# Autodesk Inventor assembly: welding-desk
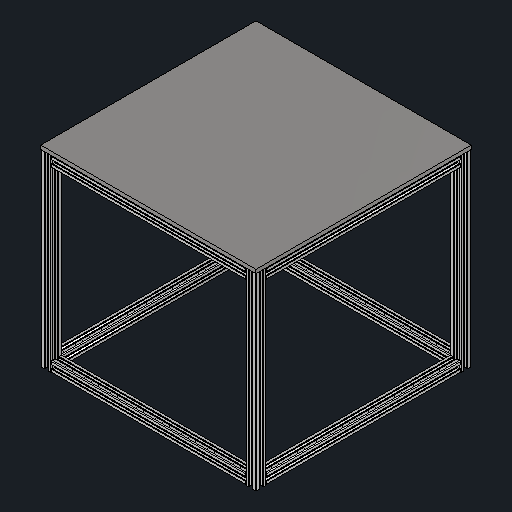
[picture p0: Inventor's stored thumbnail of the model, 512x512]
Saved by Autodesk Inventor 2026 (Build 300175050, 175E)
## iProperties
Created: 2026-01-15
Part Number: welding-desk
Document SubType Name: Assembly
Designer: queezz
Author: queezz
## Documents named in this file (5)
- C:\Users\queezz\Dropbox\Drawings\PIHTI\Desks\welding-desk.iam
- C:\Users\queezz\Dropbox\Drawings\PIHTI\Desks\welding-desk-top.ipt
- C:\Users\queezz\Dropbox\Drawings\PIHTI\ContentCenter\Aluminium-profiles\Al-profile-20x20.ipt
- C:\Users\queezz\Dropbox\Drawings\PIHTI\ContentCenter\Aluminium-profiles\Al-profile-20x20\Al-profile-20x20-360.ipt
- C:\Users\queezz\Dropbox\Drawings\PIHTI\ContentCenter\Aluminium-profiles\Al-profile-20x20\Al-profile-20x20-350.ipt
## Components (13 placed, 3 different names)
1. welding-desk-top:1 — Mate:1, Mate:2, Mate:3, Mate:4, Flush:1, Flush:2, Flush:3, Flush:4, Flush:5, Flush:6, Flush:7, Flush:8
2. Al-profile-20x20-360:1 — Mate:6, Flush:9, Flush:14, Flush:15, Flush:16
3. Al-profile-20x20-360:2 — Mate:8, Flush:11, Flush:13, Flush:14
4. Al-profile-20x20-360:3 — Mate:7, Flush:12, Flush:13
5. Al-profile-20x20-360:4 — Mate:5, Flush:10, Flush:15
6. Al-profile-20x20-360:5 — Mate:10, Flush:22, Flush:23
7. Al-profile-20x20-360:6 — Mate:12, Flush:17, Flush:20
8. Al-profile-20x20-360:7 — Mate:9, Flush:21, Flush:24
9. Al-profile-20x20-360:8 — Mate:11, Flush:18, Flush:19
10. Al-profile-20x20-350:9 — Mate:2, Flush:3, Flush:4, Mate:9, Mate:10, Flush:21, Flush:22, Flush:23, Flush:24
11. Al-profile-20x20-350:10 — Mate:3, Flush:7, Flush:8, Flush:18, Flush:19, Flush:20
12. Al-profile-20x20-350:11 — Mate:4, Flush:5, Flush:6, Mate:7, Mate:8, Flush:11, Flush:12, Mate:12, Flush:17
13. Al-profile-20x20-350:12 — Mate:1, Mate:5, Mate:6, Flush:1, Flush:2, Flush:9, Flush:10, Flush:16, Mate:11
## Relationships (36: Flush 24, Mate 12)
- Mate:1: welding-desk-top:1 ↔ Al-profile-20x20-350:12
- Mate:2: welding-desk-top:1 ↔ Al-profile-20x20-350:9
- Mate:3: welding-desk-top:1 ↔ Al-profile-20x20-350:10
- Mate:4: welding-desk-top:1 ↔ Al-profile-20x20-350:11
- Mate:5: Al-profile-20x20-360:4 ↔ Al-profile-20x20-350:12
- Mate:6: Al-profile-20x20-360:1 ↔ Al-profile-20x20-350:12
- Flush:1: welding-desk-top:1 ↔ Al-profile-20x20-350:12
- Flush:2: welding-desk-top:1 ↔ Al-profile-20x20-350:12
- Flush:3: welding-desk-top:1 ↔ Al-profile-20x20-350:9
- Flush:4: welding-desk-top:1 ↔ Al-profile-20x20-350:9
- Flush:5: welding-desk-top:1 ↔ Al-profile-20x20-350:11
- Flush:6: welding-desk-top:1 ↔ Al-profile-20x20-350:11
- Flush:7: welding-desk-top:1 ↔ Al-profile-20x20-350:10
- Flush:8: welding-desk-top:1 ↔ Al-profile-20x20-350:10
- Flush:9: Al-profile-20x20-360:1 ↔ Al-profile-20x20-350:12
- Flush:10: Al-profile-20x20-360:4 ↔ Al-profile-20x20-350:12
- Mate:7: Al-profile-20x20-360:3 ↔ Al-profile-20x20-350:11
- Mate:8: Al-profile-20x20-360:2 ↔ Al-profile-20x20-350:11
- Flush:11: Al-profile-20x20-360:2 ↔ Al-profile-20x20-350:11
- Flush:12: Al-profile-20x20-360:3 ↔ Al-profile-20x20-350:11
- Flush:13: Al-profile-20x20-360:2 ↔ Al-profile-20x20-360:3
- Flush:14: Al-profile-20x20-360:1 ↔ Al-profile-20x20-360:2
- Flush:15: Al-profile-20x20-360:1 ↔ Al-profile-20x20-360:4
- Flush:16: Al-profile-20x20-360:1 ↔ Al-profile-20x20-350:12
- Mate:9: Al-profile-20x20-360:7 ↔ Al-profile-20x20-350:9
- Mate:10: Al-profile-20x20-360:5 ↔ Al-profile-20x20-350:9
- Mate:11: Al-profile-20x20-360:8 ↔ Al-profile-20x20-350:12
- Mate:12: Al-profile-20x20-360:6 ↔ Al-profile-20x20-350:11
- Flush:17: Al-profile-20x20-360:6 ↔ Al-profile-20x20-350:11
- Flush:18: Al-profile-20x20-360:8 ↔ Al-profile-20x20-350:10
- Flush:19: Al-profile-20x20-360:8 ↔ Al-profile-20x20-350:10
- Flush:20: Al-profile-20x20-360:6 ↔ Al-profile-20x20-350:10
- Flush:21: Al-profile-20x20-360:7 ↔ Al-profile-20x20-350:9
- Flush:22: Al-profile-20x20-360:5 ↔ Al-profile-20x20-350:9
- Flush:23: Al-profile-20x20-360:5 ↔ Al-profile-20x20-350:9
- Flush:24: Al-profile-20x20-360:7 ↔ Al-profile-20x20-350:9
